# Autodesk Inventor assembly: ASY Disk Micro filter
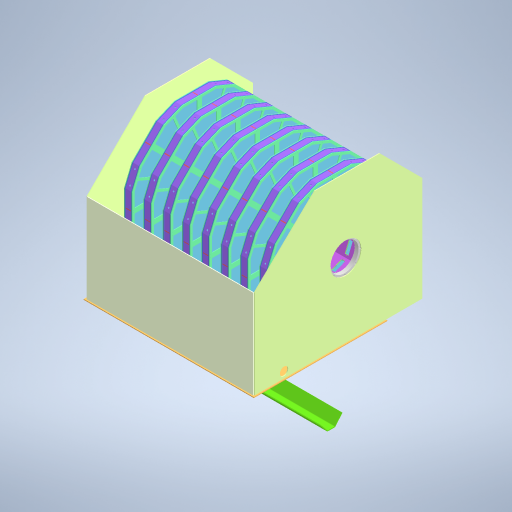
[picture p0: Inventor's stored thumbnail of the model, 512x512]
Saved by Autodesk Inventor 2024.2 (Build 282272000, 272)
## iProperties
Created: 2023-08-31
Part Number: ASY Disk Micro filter
Document SubType Name: Assembly
Designer: admin
Author: admin
## Documents named in this file (16)
- C:\Users\pokla\Documents\Inventor\ДФО\ДМФ\ДМФ 06.05.24 22-59\ДМФ 06.05.24 22-59\ASY DF Disk Micro filter.iam
- C:\Users\pokla\Documents\Inventor\ДФО\ДМФ\ДМФ 06.05.24 22-59\ДМФ 06.05.24 22-59\Left wall.ipt
- C:\Users\pokla\Documents\Inventor\ДФО\ДМФ\ДМФ 06.05.24 22-59\ДМФ 06.05.24 22-59\Wall right.ipt
- C:\Users\pokla\Documents\Inventor\ДФО\ДМФ\ДМФ 06.05.24 22-59\ДМФ 06.05.24 22-59\DF1.03 Wall bottom.ipt
- C:\Users\pokla\Documents\Inventor\ДФО\ДМФ\ДМФ 06.05.24 22-59\ДМФ 06.05.24 22-59\DF1.04 Wall face.ipt
- C:\Users\pokla\Documents\Inventor\ДФО\ДМФ\ДМФ 06.05.24 22-59\ДМФ 06.05.24 22-59\ASY DF frame.iam
- C:\Users\pokla\Documents\Inventor\ДФО\ДМФ\ДМФ 06.05.24 22-59\ДМФ 06.05.24 22-59\DF 4.1 Tray.ipt
- C:\Users\pokla\Documents\Inventor\ДФО\ДМФ\ДМФ 06.05.24 22-59\ДМФ 06.05.24 22-59\ДМС 020 кольцо прижимное 1.ipt
- C:\Users\pokla\Documents\Inventor\ДФО\ДМФ\ДМФ 06.05.24 22-59\ДМФ 06.05.24 22-59\ДМС 000 размеры.ipt
- C:\Users\pokla\Documents\Inventor\ДФО\ДМФ\ДМФ 06.05.24 22-59\ДМФ 06.05.24 22-59\ASY ДМФ 100 кольцо со шпильками.iam
- C:\Users\pokla\Documents\Inventor\ДФО\ДМФ\ДМФ 06.05.24 22-59\ДМФ 06.05.24 22-59\ДМС 040 лицо крышка.ipt
- C:\Users\pokla\Documents\Inventor\ДФО\ДМФ\ДМФ 06.05.24 22-59\ДМФ 06.05.24 22-59\ASY Вал.iam
- C:\Users\pokla\Documents\Inventor\ДФО\ДМФ\ДМФ 06.05.24 22-59\ДМФ 06.05.24 22-59\Постель 200.ipt
- C:\Users\pokla\Documents\Inventor\ДФО\ДМФ\ДМФ 06.05.24 22-59\ДМФ 06.05.24 22-59\ASY ДМФ 101 кольцо со шпильками зад.iam
- C:\Users\pokla\Documents\Inventor\ДФО\ДМФ\ДМФ 06.05.24 22-59\ДМФ 06.05.24 22-59\ДМС 021 кольцо прижимное зад.ipt
- C:\Users\pokla\Documents\Inventor\ДФО\ДМФ\ДМФ 06.05.24 22-59\ДМФ 06.05.24 22-59\Постель 201 зад.ipt
## Components (15 placed, 15 different names)
1. ДМС 000 размеры:1
2. Left wall:1 — Flush:3, Flush:4, Mate:1, Flush:6, Flush:7, Flush:9, Mate:4, Rotational:11, Flush:16, Rigid:1, Rotational:12
3. Wall right:1 — Flush:3, Mate:2, Flush:8, Rotational:14, Rotational:15
4. DF1.03 Wall bottom:1 — Mate:1, Mate:2, Flush:6, Flush:7, Flush:8, Mate:3, Flush:11, Mate:5
5. DF1.04 Wall face:1 — Flush:9, Mate:3, Mate:4, Flush:10
6. ASY DF frame:1 [sub-assembly] — Flush:15, Flush:13, Flush:14, Mate:5
7. DF 4.1 Tray:1 — Mate:7, Mate:12
8. ДМС 020 кольцо прижимное 1:1 — Rotational:12, Mate:13, Rotational:13
9. ASY ДМФ 100 кольцо со шпильками:1 [sub-assembly] — Rotational:11, Flush:16
10. ДМС 040 лицо крышка:1 — Mate:12, Rigid:1
11. ASY Вал:1 [sub-assembly] — Rotational:17
12. Постель 200:2 — Rotational:13, Flush:17, Rotational:17
13. ASY ДМФ 101 кольцо со шпильками зад:1 [sub-assembly] — Rotational:14, Mate:14
14. ДМС 021 кольцо прижимное зад:1 — Rotational:15, Flush:18, Rotational:16
15. Постель 201 зад:1 — Rotational:16, Mate:15
## Relationships (33: Flush 15, Mate 10, RevoluteJoint 7, WeldJoint 1)
- Flush:3: Left wall:1 ↔ Wall right:1
- Flush:4: Left wall:1
- Mate:1: Left wall:1 ↔ DF1.03 Wall bottom:1
- Mate:2: Wall right:1 ↔ DF1.03 Wall bottom:1
- Flush:6 (15 mm): Left wall:1 ↔ DF1.03 Wall bottom:1
- Flush:7 (25 mm): Left wall:1 ↔ DF1.03 Wall bottom:1
- Flush:8 (15 mm): Wall right:1 ↔ DF1.03 Wall bottom:1
- Flush:9: Left wall:1 ↔ DF1.04 Wall face:1
- Mate:3: DF1.03 Wall bottom:1 ↔ DF1.04 Wall face:1
- Mate:4: Left wall:1 ↔ DF1.04 Wall face:1
- Flush:10: DF1.04 Wall face:1
- Flush:11: DF1.03 Wall bottom:1
- [Flush]: ASY DF frame:1
- Flush:15: ASY DF frame:1
- Flush:13: ASY DF frame:1
- Flush:14: ASY DF frame:1
- Mate:5: DF1.03 Wall bottom:1 ↔ ASY DF frame:1
- Mate:7: DF 4.1 Tray:1
- Mate:12: DF 4.1 Tray:1 ↔ ДМС 040 лицо крышка:1
- Rotational:11 [RevoluteJoint]: Left wall:1 ↔ ASY ДМФ 100 кольцо со шпильками:1
- Flush:16: Left wall:1 ↔ ASY ДМФ 100 кольцо со шпильками:1
- Rigid:1 [WeldJoint]: Left wall:1 ↔ ДМС 040 лицо крышка:1
- Rotational:12 [RevoluteJoint]: Left wall:1 ↔ ДМС 020 кольцо прижимное 1:1
- Mate:13: ДМС 020 кольцо прижимное 1:1
- Rotational:13 [RevoluteJoint]: ДМС 020 кольцо прижимное 1:1 ↔ Постель 200:2
- Flush:17: Постель 200:2
- Rotational:14 [RevoluteJoint]: Wall right:1 ↔ ASY ДМФ 101 кольцо со шпильками зад:1
- Mate:14: ASY ДМФ 101 кольцо со шпильками зад:1
- Rotational:15 [RevoluteJoint]: Wall right:1 ↔ ДМС 021 кольцо прижимное зад:1
- Flush:18: ДМС 021 кольцо прижимное зад:1
- Rotational:16 [RevoluteJoint]: ДМС 021 кольцо прижимное зад:1 ↔ Постель 201 зад:1
- Mate:15: Постель 201 зад:1
- Rotational:17 [RevoluteJoint]: ASY Вал:1 ↔ Постель 200:2
